# Autodesk Inventor assembly: Lower 1st Stage Assembly_3rd Stage Mod
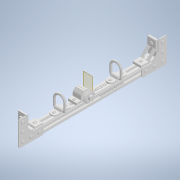
[picture p0: Inventor's stored thumbnail of the model, 180x180]
Saved by Autodesk Inventor 2020.2 (Build 242310000, 310)
## iProperties
Created: 2018-01-10
Part Number: Lower 1st Stage Assembly_3rd Stage Mod
Document SubType Name: Assembly
Designer: steele
Author: steele
Revision Number: ANY
## Documents named in this file (8)
- C:\git\CAD-Development\robSteele\2020LiftMechanism\Lower 1st Stage Assembly_3rd Stage Mod.iam
- C:\git\CAD-Development\robSteele\2020LiftMechanism\REV-21-1000 Cross member.ipt
- C:\git\CAD-Development\robSteele\2020LiftMechanism\REV-21-1002 Preloaded Assembly.iam
- C:\git\CAD-Development\robSteele\2020LiftMechanism\REV-21-1031 Preloaded Assembly.iam
- C:\git\CAD-Development\robSteele\2020LiftMechanism\REV-21-1203 Preload Assembly.iam
- C:\git\CAD-Development\robSteele\2020LiftMechanism\10-32 Slim Nylock Nut.ipt
- C:\git\CAD-Development\robSteele\2020LiftMechanism\Extra nuts.iam
- C:\git\CAD-Development\robSteele\2020LiftMechanism\Tie Down Ring.iam
## Components (17 placed, 17 different names)
1. REV-21-1000 Cross member_76
2. REV-21-1002 Preloaded Assembly_77 [sub-assembly]
3. REV-21-1002 Preloaded Assembly_78 [sub-assembly]
4. REV-21-1031 Preloaded Assembly_79 [sub-assembly]
5. REV-21-1203 Preload Assembly_80 [sub-assembly]
6. REV-21-1203 Preload Assembly_81 [sub-assembly] — Flush:1
7. 10-32 Slim Nylock Nut_82
8. 10-32 Slim Nylock Nut_83
9. 10-32 Slim Nylock Nut_84
10. 10-32 Slim Nylock Nut_85
11. 10-32 Slim Nylock Nut_86
12. 10-32 Slim Nylock Nut_87
13. 10-32 Slim Nylock Nut_88
14. 10-32 Slim Nylock Nut_89
15. Extra nuts_90 [sub-assembly]
16. Tie Down Ring_91 [sub-assembly]
17. Tie Down Ring_92 [sub-assembly]
## Relationships (1: Flush 1)
- Flush:1 (193.675 mm): REV-21-1203 Preload Assembly_81
